# Autodesk Inventor assembly: Robot Frame '16
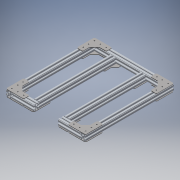
[picture p0: Inventor's stored thumbnail of the model, 180x180]
Saved by Autodesk Inventor 2017 (Build 210142000, 142)
## iProperties
Created: 2016-10-08
Part Number: Robot Frame '16
Document SubType Name: Assembly
Designer: Aditya
Author: Aditya
## Documents named in this file (7)
- C:\Users\Aditya\Documents\GitHub\RobotuxCAD\Team Robotux 15-16 Robot Cad Assets\Robot Frame '16.iam
- C:\Users\Aditya\Documents\GitHub\RobotuxCAD\Team Robotux 15-16 Robot Cad Assets\Andy Mark Parts\11.5in 1in alu ext.ipt
- C:\Users\Aditya\Documents\GitHub\RobotuxCAD\Team Robotux 15-16 Robot Cad Assets\Andy Mark Parts\15in 1in alu ext.ipt
- C:\Users\Aditya\Documents\GitHub\RobotuxCAD\Team Robotux 15-16 Robot Cad Assets\Andy Mark Parts\13in 1in alu ext.ipt
- C:\Users\Aditya\Documents\GitHub\RobotuxCAD\Team Robotux 15-16 Robot Cad Assets\Andy Mark Parts\3.7 in 1 in ext.ipt
- C:\Users\Aditya\Documents\GitHub\RobotuxCAD\Team Robotux 15-16 Robot Cad Assets\Andy Mark Parts\1in corner bracket for extrusions.ipt
- C:\Users\Aditya\Documents\GitHub\RobotuxCAD\Team Robotux 15-16 Robot Cad Assets\Andy Mark Parts\1in corner bracket for extrusions cut.ipt
## Components (19 placed, 6 different names)
1. 11.5in 1in alu ext:1 — Mate:1, Flush:1, Flush:2, Mate:2, Flush:3, Flush:4, Flush:18, Flush:20, Flush:22, Flush:25, Flush:33, Mate:18, Flush:35, Flush:38, Flush:40, Flush:50, Mate:26, Flush:51
2. 15in 1in alu ext:1 — Mate:2, Flush:3, Flush:4, Mate:4, Flush:7, Flush:8, Mate:8, Flush:16, Mate:9, Flush:17, Mate:11, Flush:21, Mate:12, Flush:24, Mate:23, Flush:46, Mate:24, Flush:47, Mate:25, Flush:49, Flush:52
3. 15in 1in alu ext:2 — Mate:1, Flush:1, Flush:2, Mate:3, Flush:5, Flush:6, Mate:7, Flush:14, Mate:10, Flush:19, Mate:13, Flush:26, Mate:14, Flush:28, Mate:19, Flush:37, Mate:20, Flush:39, Mate:21, Flush:41, Flush:44
4. 13in 1in alu ext:1 — Mate:5, Flush:9, Flush:10, Flush:32, Mate:17, Flush:34
5. 13in 1in alu ext:2 — Mate:6, Flush:11, Flush:12, Mate:15, Flush:30, Flush:36
6. 3.7 in 1 in ext:1 — Mate:4, Flush:7, Flush:8, Mate:5, Flush:9, Flush:10, Flush:15, Flush:23, Mate:16, Flush:31, Flush:45, Flush:48
7. 3.7 in 1 in ext:2 — Mate:3, Flush:5, Flush:6, Mate:6, Flush:11, Flush:12, Flush:13, Flush:27, Flush:29, Flush:42, Mate:22, Flush:43
8. 1in corner bracket for extrusions:1 — Mate:10, Flush:19, Flush:20, Mate:20, Flush:39, Flush:40
9. 1in corner bracket for extrusions:2 — Mate:8, Flush:15, Flush:16, Mate:24, Flush:47, Flush:48
10. 1in corner bracket for extrusions:3 — Mate:7, Flush:13, Flush:14, Mate:22, Flush:43, Flush:44
11. 1in corner bracket for extrusions:4 — Mate:9, Flush:17, Flush:18, Mate:26, Flush:51, Flush:52
12. 1in corner bracket for extrusions:5 — Mate:11, Flush:21, Flush:22, Mate:25, Flush:49, Flush:50
13. 1in corner bracket for extrusions:6 — Mate:13, Flush:25, Flush:26, Mate:19, Flush:37, Flush:38
14. 1in corner bracket for extrusions:7 — Mate:14, Flush:27, Flush:28, Mate:21, Flush:41, Flush:42
15. 1in corner bracket for extrusions:8 — Mate:12, Flush:23, Flush:24, Mate:23, Flush:45, Flush:46
16. 1in corner bracket for extrusions cut:1 — Mate:17, Flush:33, Flush:34
17. 1in corner bracket for extrusions cut:2 — Mate:15, Flush:29, Flush:30
18. 1in corner bracket for extrusions cut:3 — Mate:18, Flush:35, Flush:36
19. 1in corner bracket for extrusions cut:4 — Mate:16, Flush:31, Flush:32
## Relationships (78: Flush 52, Mate 26)
- Mate:1: 11.5in 1in alu ext:1 ↔ 15in 1in alu ext:2
- Flush:1: 11.5in 1in alu ext:1 ↔ 15in 1in alu ext:2
- Flush:2: 11.5in 1in alu ext:1 ↔ 15in 1in alu ext:2
- Mate:2: 11.5in 1in alu ext:1 ↔ 15in 1in alu ext:1
- Flush:3: 11.5in 1in alu ext:1 ↔ 15in 1in alu ext:1
- Flush:4: 11.5in 1in alu ext:1 ↔ 15in 1in alu ext:1
- Mate:3: 15in 1in alu ext:2 ↔ 3.7 in 1 in ext:2
- Flush:5: 15in 1in alu ext:2 ↔ 3.7 in 1 in ext:2
- Flush:6: 15in 1in alu ext:2 ↔ 3.7 in 1 in ext:2
- Mate:4: 15in 1in alu ext:1 ↔ 3.7 in 1 in ext:1
- Flush:7: 15in 1in alu ext:1 ↔ 3.7 in 1 in ext:1
- Flush:8: 15in 1in alu ext:1 ↔ 3.7 in 1 in ext:1
- Mate:5: 13in 1in alu ext:1 ↔ 3.7 in 1 in ext:1
- Flush:9: 13in 1in alu ext:1 ↔ 3.7 in 1 in ext:1
- Flush:10: 13in 1in alu ext:1 ↔ 3.7 in 1 in ext:1
- Mate:6: 13in 1in alu ext:2 ↔ 3.7 in 1 in ext:2
- Flush:11: 13in 1in alu ext:2 ↔ 3.7 in 1 in ext:2
- Flush:12: 13in 1in alu ext:2 ↔ 3.7 in 1 in ext:2
- Mate:7: 15in 1in alu ext:2 ↔ 1in corner bracket for extrusions:3
- Flush:13: 3.7 in 1 in ext:2 ↔ 1in corner bracket for extrusions:3
- Flush:14: 15in 1in alu ext:2 ↔ 1in corner bracket for extrusions:3
- Mate:8: 15in 1in alu ext:1 ↔ 1in corner bracket for extrusions:2
- Flush:15: 3.7 in 1 in ext:1 ↔ 1in corner bracket for extrusions:2
- Flush:16: 15in 1in alu ext:1 ↔ 1in corner bracket for extrusions:2
- Mate:9: 15in 1in alu ext:1 ↔ 1in corner bracket for extrusions:4
- Flush:17: 15in 1in alu ext:1 ↔ 1in corner bracket for extrusions:4
- Flush:18: 11.5in 1in alu ext:1 ↔ 1in corner bracket for extrusions:4
- Mate:10: 15in 1in alu ext:2 ↔ 1in corner bracket for extrusions:1
- Flush:19: 15in 1in alu ext:2 ↔ 1in corner bracket for extrusions:1
- Flush:20: 11.5in 1in alu ext:1 ↔ 1in corner bracket for extrusions:1
- Mate:11: 15in 1in alu ext:1 ↔ 1in corner bracket for extrusions:5
- Flush:21: 15in 1in alu ext:1 ↔ 1in corner bracket for extrusions:5
- Flush:22: 11.5in 1in alu ext:1 ↔ 1in corner bracket for extrusions:5
- Mate:12: 15in 1in alu ext:1 ↔ 1in corner bracket for extrusions:8
- Flush:23: 3.7 in 1 in ext:1 ↔ 1in corner bracket for extrusions:8
- Flush:24: 15in 1in alu ext:1 ↔ 1in corner bracket for extrusions:8
- Mate:13: 15in 1in alu ext:2 ↔ 1in corner bracket for extrusions:6
- Flush:25: 11.5in 1in alu ext:1 ↔ 1in corner bracket for extrusions:6
- Flush:26: 15in 1in alu ext:2 ↔ 1in corner bracket for extrusions:6
- Mate:14: 15in 1in alu ext:2 ↔ 1in corner bracket for extrusions:7
- Flush:27: 3.7 in 1 in ext:2 ↔ 1in corner bracket for extrusions:7
- Flush:28: 15in 1in alu ext:2 ↔ 1in corner bracket for extrusions:7
- Mate:15: 13in 1in alu ext:2 ↔ 1in corner bracket for extrusions cut:2
- Flush:29: 3.7 in 1 in ext:2 ↔ 1in corner bracket for extrusions cut:2
- Flush:30: 13in 1in alu ext:2 ↔ 1in corner bracket for extrusions cut:2
- Mate:16: 3.7 in 1 in ext:1 ↔ 1in corner bracket for extrusions cut:4
- Flush:31: 3.7 in 1 in ext:1 ↔ 1in corner bracket for extrusions cut:4
- Flush:32: 13in 1in alu ext:1 ↔ 1in corner bracket for extrusions cut:4
- Mate:17: 13in 1in alu ext:1 ↔ 1in corner bracket for extrusions cut:1
- Flush:33: 11.5in 1in alu ext:1 ↔ 1in corner bracket for extrusions cut:1
- Flush:34: 13in 1in alu ext:1 ↔ 1in corner bracket for extrusions cut:1
- Mate:18: 11.5in 1in alu ext:1 ↔ 1in corner bracket for extrusions cut:3
- Flush:35: 11.5in 1in alu ext:1 ↔ 1in corner bracket for extrusions cut:3
- Flush:36: 13in 1in alu ext:2 ↔ 1in corner bracket for extrusions cut:3
- Mate:19: 15in 1in alu ext:2 ↔ 1in corner bracket for extrusions:6
- Flush:37: 15in 1in alu ext:2 ↔ 1in corner bracket for extrusions:6
- Flush:38: 11.5in 1in alu ext:1 ↔ 1in corner bracket for extrusions:6
- Mate:20: 15in 1in alu ext:2 ↔ 1in corner bracket for extrusions:1
- Flush:39: 15in 1in alu ext:2 ↔ 1in corner bracket for extrusions:1
- Flush:40: 11.5in 1in alu ext:1 ↔ 1in corner bracket for extrusions:1
- Mate:21: 15in 1in alu ext:2 ↔ 1in corner bracket for extrusions:7
- Flush:41: 15in 1in alu ext:2 ↔ 1in corner bracket for extrusions:7
- Flush:42: 3.7 in 1 in ext:2 ↔ 1in corner bracket for extrusions:7
- Mate:22: 3.7 in 1 in ext:2 ↔ 1in corner bracket for extrusions:3
- Flush:43: 3.7 in 1 in ext:2 ↔ 1in corner bracket for extrusions:3
- Flush:44: 15in 1in alu ext:2 ↔ 1in corner bracket for extrusions:3
- Mate:23: 15in 1in alu ext:1 ↔ 1in corner bracket for extrusions:8
- Flush:45: 3.7 in 1 in ext:1 ↔ 1in corner bracket for extrusions:8
- Flush:46: 15in 1in alu ext:1 ↔ 1in corner bracket for extrusions:8
- Mate:24: 15in 1in alu ext:1 ↔ 1in corner bracket for extrusions:2
- Flush:47: 15in 1in alu ext:1 ↔ 1in corner bracket for extrusions:2
- Flush:48: 3.7 in 1 in ext:1 ↔ 1in corner bracket for extrusions:2
- Mate:25: 15in 1in alu ext:1 ↔ 1in corner bracket for extrusions:5
- Flush:49: 15in 1in alu ext:1 ↔ 1in corner bracket for extrusions:5
- Flush:50: 11.5in 1in alu ext:1 ↔ 1in corner bracket for extrusions:5
- Mate:26: 11.5in 1in alu ext:1 ↔ 1in corner bracket for extrusions:4
- Flush:51: 11.5in 1in alu ext:1 ↔ 1in corner bracket for extrusions:4
- Flush:52: 15in 1in alu ext:1 ↔ 1in corner bracket for extrusions:4
